# Autodesk Inventor assembly: RT_FRM_A_002
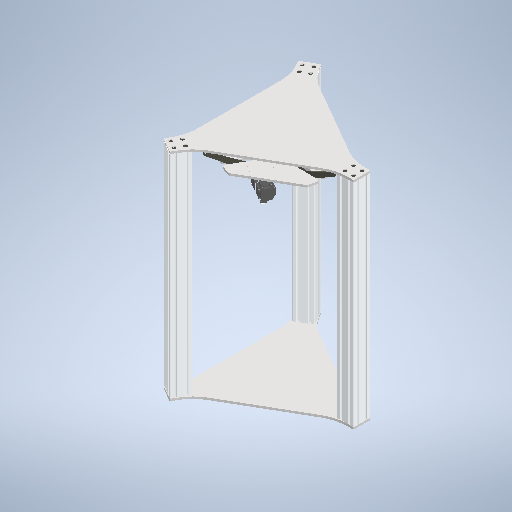
[picture p0: Inventor's stored thumbnail of the model, 512x512]
Saved by Autodesk Inventor 2025.3 (Build 293356000, 356)
## iProperties
Created: 2026-05-11
Part Number: RT_FRM_A_002
Document SubType Name: Assembly
Designer: louis
Author: louis
## Documents named in this file (6)
- C:\Users\louis\OneDrive\Desktop\R_Trident\02_CAD\04_Subassemblies\RT_FRM_A_002.iam
- C:\Users\louis\OneDrive\Desktop\R_Trident\02_CAD\03_Parts_Custom\RT_FRM_MC_004_TopPlate.ipt
- C:\Users\louis\OneDrive\Desktop\R_Trident\02_CAD\04_Subassemblies\RT_ARM_A_001.iam
- C:\Users\louis\OneDrive\Desktop\R_Trident\02_CAD\03_Parts_Custom\RT_FRM_MC_004_BasePlateTop.ipt
- C:\Users\louis\OneDrive\Desktop\R_Trident\02_CAD\01_Standard_Parts\3699_20251009135551_8080x100\3699_20251009135551_8080x100\3699_20251009135551_8080x100.ipt
- C:\Users\louis\OneDrive\Documents\Inventor\Content Center Files\R2025\en-US\ISO 10642(1)\ISO 10642 - M8 x  25.ipt
## Components (33 placed, 5 different names)
1. RT_FRM_MC_004_TopPlate:1 — Mate:1, Flush:3, Mate:3, Mate:4, Mate:5, Mate:6, Mate:7, Mate:8, Mate:9, Mate:26
2. RT_ARM_A_001:1 [sub-assembly] — Mate:4, Mate:5, Mate:14
3. RT_ARM_A_001:2 [sub-assembly] — Mate:6, Mate:7, Mate:15
4. RT_ARM_A_001:3 [sub-assembly] — Mate:8, Mate:9, Mate:16
5. 3699_20251009135551_8080x100:1 — Mate:24, Mate:25
6. 3699_20251009135551_8080x100:2 — Mate:22, Mate:23
7. 3699_20251009135551_8080x100:3 — Mate:20, Mate:21, Mate:27, Mate:28
8. RT_FRM_MC_004_BasePlateTop:1 — Mate:19, Flush:4, Mate:20, Mate:21, Mate:22, Mate:23, Mate:24, Mate:25, Mate:26, Mate:29, Mate:30, Mate:31, Mate:32, Mate:33, Mate:34, Mate:35, Mate:36, Mate:37, Mate:38, Mate:39, Mate:40
9. RT_FRM_MC_004_BasePlateTop:2 — Mate:27, Mate:28, Mate:41, Mate:42, Mate:43, Mate:44, Mate:45, Mate:46, Mate:47, Mate:48, Mate:49, Mate:50, Mate:51, Mate:52
10. ISO 10642 M8x25:1 — Mate:29
11. ISO 10642 M8x25:2 — Mate:30
12. ISO 10642 M8x25:3 — Mate:31
13. ISO 10642 M8x25:4 — Mate:32
14. ISO 10642 M8x25:5 — Mate:33
15. ISO 10642 M8x25:6 — Mate:34
16. ISO 10642 M8x25:7 — Mate:35
17. ISO 10642 M8x25:8 — Mate:36
18. ISO 10642 M8x25:9 — Mate:37
19. ISO 10642 M8x25:10 — Mate:38
20. ISO 10642 M8x25:11 — Mate:39
21. ISO 10642 M8x25:12 — Mate:40
22. ISO 10642 M8x25:13 — Mate:41
23. ISO 10642 M8x25:14 — Mate:42
24. ISO 10642 M8x25:15 — Mate:43
25. ISO 10642 M8x25:16 — Mate:44
26. ISO 10642 M8x25:17 — Mate:45
27. ISO 10642 M8x25:18 — Mate:46
28. ISO 10642 M8x25:19 — Mate:47
29. ISO 10642 M8x25:20 — Mate:48
30. ISO 10642 M8x25:21 — Mate:49
31. ISO 10642 M8x25:22 — Mate:50
32. ISO 10642 M8x25:23 — Mate:51
33. ISO 10642 M8x25:24 — Mate:52
## Relationships (48: Mate 45, Flush 3)
- Mate:1: RT_FRM_MC_004_TopPlate:1
- Flush:3: RT_FRM_MC_004_TopPlate:1
- Mate:3: RT_FRM_MC_004_TopPlate:1
- Mate:4: RT_FRM_MC_004_TopPlate:1 ↔ RT_ARM_A_001:1
- Mate:5: RT_FRM_MC_004_TopPlate:1 ↔ RT_ARM_A_001:1
- Mate:6: RT_FRM_MC_004_TopPlate:1 ↔ RT_ARM_A_001:2
- Mate:7: RT_FRM_MC_004_TopPlate:1 ↔ RT_ARM_A_001:2
- Mate:8: RT_FRM_MC_004_TopPlate:1 ↔ RT_ARM_A_001:3
- Mate:9: RT_FRM_MC_004_TopPlate:1 ↔ RT_ARM_A_001:3
- Mate:14: RT_ARM_A_001:1
- Mate:15: RT_ARM_A_001:2
- Mate:16: RT_ARM_A_001:3
- Flush:1 (700 mm)
- Mate:19: RT_FRM_MC_004_BasePlateTop:1
- Flush:4: RT_FRM_MC_004_BasePlateTop:1
- Mate:20: 3699_20251009135551_8080x100:3 ↔ RT_FRM_MC_004_BasePlateTop:1
- Mate:21: 3699_20251009135551_8080x100:3 ↔ RT_FRM_MC_004_BasePlateTop:1
- Mate:22: 3699_20251009135551_8080x100:2 ↔ RT_FRM_MC_004_BasePlateTop:1
- Mate:23: 3699_20251009135551_8080x100:2 ↔ RT_FRM_MC_004_BasePlateTop:1
- Mate:24: 3699_20251009135551_8080x100:1 ↔ RT_FRM_MC_004_BasePlateTop:1
- Mate:25: 3699_20251009135551_8080x100:1 ↔ RT_FRM_MC_004_BasePlateTop:1
- Mate:26 (100 mm): RT_FRM_MC_004_TopPlate:1 ↔ RT_FRM_MC_004_BasePlateTop:1
- Mate:27: 3699_20251009135551_8080x100:3 ↔ RT_FRM_MC_004_BasePlateTop:2
- Mate:28: 3699_20251009135551_8080x100:3 ↔ RT_FRM_MC_004_BasePlateTop:2
- Mate:29: RT_FRM_MC_004_BasePlateTop:1 ↔ ISO 10642 M8x25:1
- Mate:30: RT_FRM_MC_004_BasePlateTop:1 ↔ ISO 10642 M8x25:2
- Mate:31: RT_FRM_MC_004_BasePlateTop:1 ↔ ISO 10642 M8x25:3
- Mate:32: RT_FRM_MC_004_BasePlateTop:1 ↔ ISO 10642 M8x25:4
- Mate:33: RT_FRM_MC_004_BasePlateTop:1 ↔ ISO 10642 M8x25:5
- Mate:34: RT_FRM_MC_004_BasePlateTop:1 ↔ ISO 10642 M8x25:6
- Mate:35: RT_FRM_MC_004_BasePlateTop:1 ↔ ISO 10642 M8x25:7
- Mate:36: RT_FRM_MC_004_BasePlateTop:1 ↔ ISO 10642 M8x25:8
- Mate:37: RT_FRM_MC_004_BasePlateTop:1 ↔ ISO 10642 M8x25:9
- Mate:38: RT_FRM_MC_004_BasePlateTop:1 ↔ ISO 10642 M8x25:10
- Mate:39: RT_FRM_MC_004_BasePlateTop:1 ↔ ISO 10642 M8x25:11
- Mate:40: RT_FRM_MC_004_BasePlateTop:1 ↔ ISO 10642 M8x25:12
- Mate:41: RT_FRM_MC_004_BasePlateTop:2 ↔ ISO 10642 M8x25:13
- Mate:42: RT_FRM_MC_004_BasePlateTop:2 ↔ ISO 10642 M8x25:14
- Mate:43: RT_FRM_MC_004_BasePlateTop:2 ↔ ISO 10642 M8x25:15
- Mate:44: RT_FRM_MC_004_BasePlateTop:2 ↔ ISO 10642 M8x25:16
- Mate:45: RT_FRM_MC_004_BasePlateTop:2 ↔ ISO 10642 M8x25:17
- Mate:46: RT_FRM_MC_004_BasePlateTop:2 ↔ ISO 10642 M8x25:18
- Mate:47: RT_FRM_MC_004_BasePlateTop:2 ↔ ISO 10642 M8x25:19
- Mate:48: RT_FRM_MC_004_BasePlateTop:2 ↔ ISO 10642 M8x25:20
- Mate:49: RT_FRM_MC_004_BasePlateTop:2 ↔ ISO 10642 M8x25:21
- Mate:50: RT_FRM_MC_004_BasePlateTop:2 ↔ ISO 10642 M8x25:22
- Mate:51: RT_FRM_MC_004_BasePlateTop:2 ↔ ISO 10642 M8x25:23
- Mate:52: RT_FRM_MC_004_BasePlateTop:2 ↔ ISO 10642 M8x25:24
